# Autodesk Inventor assembly: 四个白垫片
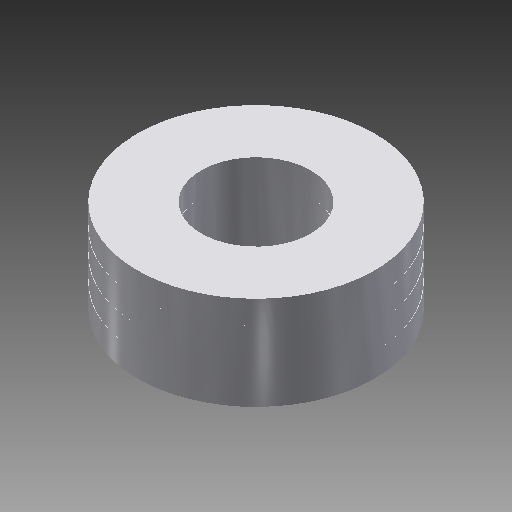
[picture p0: Inventor's stored thumbnail of the model, 512x512]
Saved by Autodesk Inventor 2019.3 (Build 233278000, 278)
## iProperties
Created: 2019-03-26
Part Number: 四个白垫片
Material: 常规
Document SubType Name: Assembly
Designer: aresp
Mass: 0.223507 g
Surface Area: 6.13108 cm^2
Volume: 0.210855 cm^3
Density: 1.06 g/cm^3
Author: aresp
## Documents named in this file (2)
- D:\cad\零件库\四个白垫片.iam
- D:\cad\零件库\垫片轴套大白等\Washer, Delrin, 0.04''.ipt
## Components (4 placed, 1 different names)
1. Washer, Delrin, 0.04'':1
2. Washer, Delrin, 0.04'':2
3. Washer, Delrin, 0.04'':3
4. Washer, Delrin, 0.04'':4
## Relationships (6: Mate 6)
- [Mate]: Washer, Delrin, 0.04'':3 ↔ Washer, Delrin, 0.04'':4
- [Mate]: Washer, Delrin, 0.04'':1 ↔ Washer, Delrin, 0.04'':4
- [Mate]: Washer, Delrin, 0.04'':2 ↔ Washer, Delrin, 0.04'':4
- [Mate]: Washer, Delrin, 0.04'':2 ↔ Washer, Delrin, 0.04'':3
- [Mate]: Washer, Delrin, 0.04'':2 ↔ Washer, Delrin, 0.04'':4
- [Mate]: Washer, Delrin, 0.04'':1 ↔ Washer, Delrin, 0.04'':4
